# Autodesk Inventor assembly: Coupler lift long with bracket
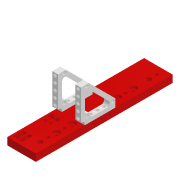
[picture p0: Inventor's stored thumbnail of the model, 180x180]
Saved by Autodesk Inventor 2020 (Build 240168000, 168)
## iProperties
Created: 2019-11-25
Part Number: Coupler lift long with bracket
Document SubType Name: Assembly
Designer: ball
Author: ball
## Documents named in this file (3)
- C:\FTC\FTC8863CAD\2019 Robot\Delivery\Coupler lift long with bracket.iam
- C:\FTC\FTC8863CAD\2019 Robot\Delivery\Coupler lift long with bracket.ipt
- C:\FTC\FTC8863CAD\GoBilda\1204 Parts\1204-0002-0001.ipt
## Components (3 placed, 2 different names)
1. Coupler lift long with bracket:1 — Mate:1, Flush:1, Flush:2, Mate:2, Flush:3, Flush:4
2. 1204-0002-0001:1 — Mate:1, Flush:1, Flush:2
3. 1204-0002-0001:2 — Mate:2, Flush:3, Flush:4
## Relationships (6: Flush 4, Mate 2)
- Mate:1: Coupler lift long with bracket:1 ↔ 1204-0002-0001:1
- Flush:1: Coupler lift long with bracket:1 ↔ 1204-0002-0001:1
- Flush:2 (55.88 mm): Coupler lift long with bracket:1 ↔ 1204-0002-0001:1
- Mate:2: Coupler lift long with bracket:1 ↔ 1204-0002-0001:2
- Flush:3 (55.88 mm): Coupler lift long with bracket:1 ↔ 1204-0002-0001:2
- Flush:4: Coupler lift long with bracket:1 ↔ 1204-0002-0001:2
